# Autodesk Inventor assembly: board_set
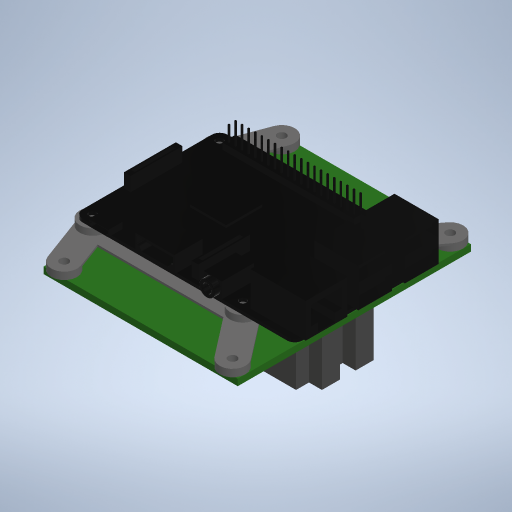
[picture p0: Inventor's stored thumbnail of the model, 512x512]
Saved by Autodesk Inventor 2024.1 (Build 281209000, 209)
## iProperties
Created: 2024-08-02
Part Number: board_set
Document SubType Name: Assembly
Designer: hibik
Author: hibik
## Documents named in this file (4)
- C:\Users\hibik\Desktop\ロボメカ\Rescue\2年\子機_本選\board_set.iam
- C:\Users\hibik\Desktop\ロボメカ\Rescue\2年\子機_本選\board_connector.ipt
- C:\Users\hibik\Desktop\ロボメカ\Rescue\2年\子機_本選\control_board.ipt
- C:\Users\hibik\Desktop\ロボメカ\Rescue\2年\子機_本選\Raspberrypi3.ipt
## Components (3 placed, 3 different names)
1. board_connector:1 — 挿入:1, 挿入:2, 挿入:3, 挿入:4
2. control_board:1 — 挿入:3, 挿入:4
3. Raspberrypi3:1 — 挿入:1, 挿入:2
## Relationships (4: Insert 4)
- 挿入:1 [Insert]: board_connector:1 ↔ Raspberrypi3:1
- 挿入:2 [Insert]: board_connector:1 ↔ Raspberrypi3:1
- 挿入:3 [Insert]: board_connector:1 ↔ control_board:1
- 挿入:4 [Insert]: board_connector:1 ↔ control_board:1
